# Autodesk Inventor assembly: FullAssembly
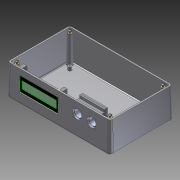
[picture p0: Inventor's stored thumbnail of the model, 180x180]
Saved by Autodesk Inventor 2015 (Build 190159000, 159)
## iProperties
Created: 2015-03-06
Part Number: FullAssembly
Document SubType Name: Assembly
Designer: ChristopherEvan
Author: ChristopherEvan
## Documents named in this file (4)
- C:\Users\ChristopherEvan\Documents\Inventor\MAKE\FullAssembly.iam
- C:\Users\ChristopherEvan\Documents\Inventor\MAKE\Enclosure\Enclosure.iam
- C:\Users\ChristopherEvan\Documents\Inventor\MAKE\Enclosure\ProxSensor\hc-sr04.iam
- C:\Users\ChristopherEvan\Documents\Inventor\MAKE\Enclosure\LCD\LCD_with_bracket.iam
## Components (3 placed, 3 different names)
1. Enclosure:1 [sub-assembly] — Mate:1, Mate:2
2. hc-sr04:1 [sub-assembly] — Mate:1
3. LCD_with_bracket:1 [sub-assembly] — Mate:2
## Relationships (2: Mate 2)
- Mate:1: Enclosure:1 ↔ hc-sr04:1
- Mate:2: Enclosure:1 ↔ LCD_with_bracket:1
